# Autodesk Inventor assembly: complete mount for leica brick
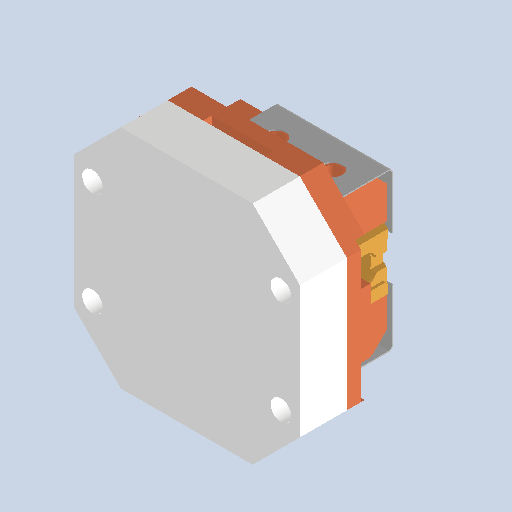
[picture p0: Inventor's stored thumbnail of the model, 512x512]
Saved by Autodesk Inventor 2026.1 (Build 301233000, 233)
## iProperties
Created: 2023-04-19
Part Number: complete mount for leica brick
Document SubType Name: Assembly
Designer: Julian
Author: Julian
## Documents named in this file (5)
- C:\Users\user\Desktop\setup_inventor_2025\single-objective\sample mount for lego brick\complete mount for leica brick.iam
- C:\Users\user\Desktop\setup_inventor_2025\single-objective\sample mount for lego brick\marcor_isolator.ipt
- C:\Users\user\Desktop\setup_inventor_2025\single-objective\sample mount for lego brick\ProbenhalterungKasette.ipt
- C:\Users\user\Desktop\setup_inventor_2025\single-objective\sample mount for lego brick\Clmap for sample mount for new Leica System.ipt
- C:\Users\user\Desktop\setup_inventor_2025\single-objective\CLEM Cartridge gespannte Feder_ipt.iam
## Components (5 placed, 4 different names)
1. marcor_isolator:1 — Mate:1, Mate:2, Mate:3
2. ProbenhalterungKasette:1 — Mate:1, Mate:2, Mate:3, Mate:4, Mate:5, Mate:6, Mate:7, Mate:8, Mate:9, Passend:10, Passend:11, Passend:12
3. Clmap for sample mount for new Leica System:1 — Mate:4, Mate:5, Mate:6
4. Clmap for sample mount for new Leica System:2 — Mate:7, Mate:8, Mate:9
5. CLEM Cartridge gespannte Feder_ipt:1 [sub-assembly] — Passend:10, Passend:11, Passend:12
## Relationships (12: Mate 12)
- Mate:1: marcor_isolator:1 ↔ ProbenhalterungKasette:1
- Mate:2: marcor_isolator:1 ↔ ProbenhalterungKasette:1
- Mate:3: marcor_isolator:1 ↔ ProbenhalterungKasette:1
- Mate:4: ProbenhalterungKasette:1 ↔ Clmap for sample mount for new Leica System:1
- Mate:5: ProbenhalterungKasette:1 ↔ Clmap for sample mount for new Leica System:1
- Mate:6: ProbenhalterungKasette:1 ↔ Clmap for sample mount for new Leica System:1
- Mate:7: ProbenhalterungKasette:1 ↔ Clmap for sample mount for new Leica System:2
- Mate:8: ProbenhalterungKasette:1 ↔ Clmap for sample mount for new Leica System:2
- Mate:9: ProbenhalterungKasette:1 ↔ Clmap for sample mount for new Leica System:2
- Passend:10 [Mate]: ProbenhalterungKasette:1 ↔ CLEM Cartridge gespannte Feder_ipt:1
- Passend:11 [Mate] (0.25 mm): ProbenhalterungKasette:1 ↔ CLEM Cartridge gespannte Feder_ipt:1
- Passend:12 [Mate]: ProbenhalterungKasette:1 ↔ CLEM Cartridge gespannte Feder_ipt:1
